# Autodesk Inventor assembly: Marina - simplificacion
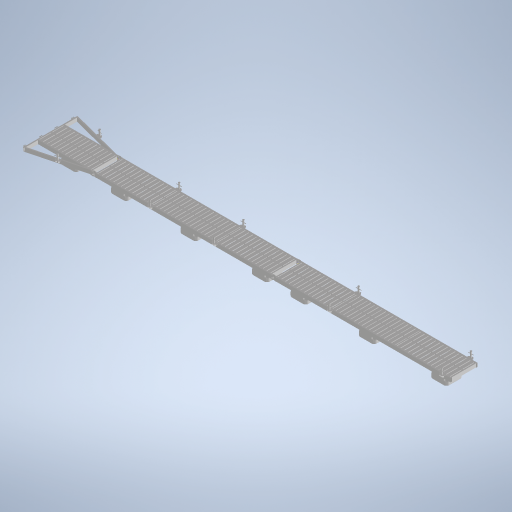
[picture p0: Inventor's stored thumbnail of the model, 512x512]
Saved by Autodesk Inventor 2023.2 (Build 272271000, 271)
## iProperties
Created: 2022-11-23
Part Number: Marina - simplificacion
Document SubType Name: Assembly
Designer: Maestria 1
Author: Maestria 1
## Documents named in this file (3)
- C:\Users\nekko\Documents\Modelos Orza SpA\Marina - simplificacion.iam
- C:\Users\nekko\Documents\Modelos Orza SpA\armazon.ipt
- C:\Users\nekko\Documents\Modelos Orza SpA\peldaño.ipt
## Components (103 placed, 2 different names)
1. armazon:1 — Nivelación:1, Coincidencia:1, Coincidencia:2, Nivelación:2, Coincidencia:3, Coincidencia:4, Coincidencia:5, Nivelación:3, Coincidencia:6, Mate:7, Flush:4, Mate:8, Flush:6, Flush:7, Mate:9, Flush:8, Mate:10, Flush:10, Flush:11, Mate:11, Flush:12, Mate:12, Flush:14, Flush:15, Mate:13, Flush:16, Mate:14, Flush:18, Flush:19, Flush:20, Mate:15, Mate:17, Flush:21, Flush:22, Mate:18, Flush:23
2. peldaño:2 — Nivelación:1, Coincidencia:1, Coincidencia:2
3. peldaño:1 — Nivelación:2, Coincidencia:3, Coincidencia:4
4. peldaño:15
5. peldaño:16
6. peldaño:17
7. peldaño:18
8. peldaño:19
9. peldaño:20
10. peldaño:21
11. peldaño:22
12. peldaño:23
13. peldaño:24
14. peldaño:25
15. peldaño:26
16. peldaño:3 — Mate:7, Flush:4, Flush:5
17. peldaño:4 — Coincidencia:5, Nivelación:3, Coincidencia:6, Flush:5
18. peldaño:27
19. peldaño:28
20. peldaño:29
21. peldaño:30
22. peldaño:31
23. peldaño:32
24. peldaño:33
25. peldaño:34
26. peldaño:35
27. peldaño:36
28. peldaño:37
29. peldaño:38
30. peldaño:7 — Mate:8, Flush:6, Flush:7, Flush:9
31. peldaño:6 — Mate:9, Flush:8, Flush:9
32. peldaño:39
33. peldaño:40
34. peldaño:41
35. peldaño:42
36. peldaño:43
37. peldaño:44
38. peldaño:45
39. peldaño:46
40. peldaño:47
41. peldaño:48
42. peldaño:49
43. peldaño:50
44. peldaño:51
45. peldaño:52
46. peldaño:5 — Mate:10, Flush:10, Flush:11, Flush:13
47. peldaño:8 — Mate:11, Flush:12, Flush:13
48. peldaño:53
49. peldaño:54
50. peldaño:55
51. peldaño:56
52. peldaño:57
53. peldaño:58
54. peldaño:59
55. peldaño:60
56. peldaño:61
57. peldaño:62
58. peldaño:63
59. peldaño:64
60. peldaño:9 — Mate:12, Flush:14, Flush:15, Flush:17
61. peldaño:10 — Mate:13, Flush:16, Flush:17
62. peldaño:65
63. peldaño:66
64. peldaño:67
65. peldaño:68
66. peldaño:69
67. peldaño:70
68. peldaño:71
69. peldaño:72
70. peldaño:73
71. peldaño:74
72. peldaño:75
73. peldaño:76
74. peldaño:11 — Flush:20, Mate:15, Mate:16
75. peldaño:12 — Mate:14, Flush:18, Flush:19, Mate:16
76. peldaño:77
77. peldaño:78
78. peldaño:79
79. peldaño:80
80. peldaño:81
81. peldaño:82
82. peldaño:83
83. peldaño:84
84. peldaño:85
85. peldaño:86
86. peldaño:87
87. peldaño:88
88. peldaño:89
89. peldaño:90
90. peldaño:13 — Mate:18, Flush:23, Flush:24
91. peldaño:14 — Mate:17, Flush:21, Flush:22, Flush:24
92. peldaño:91
93. peldaño:92
94. peldaño:93
95. peldaño:94
96. peldaño:95
97. peldaño:96
98. peldaño:97
99. peldaño:98
100. peldaño:99
101. peldaño:100
102. peldaño:101
103. peldaño:102
## Component patterns: (7 elements, first: peldaño:2 + peldaño:1), (7 elements, first: peldaño:3 + peldaño:4), (8 elements, first: peldaño:7 + peldaño:6), (7 elements, first: peldaño:5 + peldaño:8), (7 elements, first: peldaño:9 + peldaño:10), (8 elements, first: peldaño:11 + peldaño:12), (7 elements, first: peldaño:13 + peldaño:14)
## Relationships (42: Flush 24, Mate 18)
- Nivelación:1 [Flush]: armazon:1 ↔ peldaño:2
- Coincidencia:1 [Mate]: armazon:1 ↔ peldaño:2
- Coincidencia:2 [Mate] (25 mm): armazon:1 ↔ peldaño:2
- Nivelación:2 [Flush]: armazon:1 ↔ peldaño:1
- Coincidencia:3 [Mate]: armazon:1 ↔ peldaño:1
- Coincidencia:4 [Mate] (25 mm): armazon:1 ↔ peldaño:1
- Coincidencia:5 [Mate]: armazon:1 ↔ peldaño:4
- Nivelación:3 [Flush]: armazon:1 ↔ peldaño:4
- Coincidencia:6 [Mate] (25 mm): armazon:1 ↔ peldaño:4
- Mate:7: armazon:1 ↔ peldaño:3
- Flush:4: armazon:1 ↔ peldaño:3
- Flush:5: peldaño:3 ↔ peldaño:4
- Mate:8: armazon:1 ↔ peldaño:7
- Flush:6: armazon:1 ↔ peldaño:7
- Flush:7 (25 mm): armazon:1 ↔ peldaño:7
- Mate:9: armazon:1 ↔ peldaño:6
- Flush:8: armazon:1 ↔ peldaño:6
- Flush:9: peldaño:7 ↔ peldaño:6
- Mate:10: armazon:1 ↔ peldaño:5
- Flush:10: armazon:1 ↔ peldaño:5
- Flush:11 (25 mm): armazon:1 ↔ peldaño:5
- Mate:11: armazon:1 ↔ peldaño:8
- Flush:12: armazon:1 ↔ peldaño:8
- Flush:13: peldaño:5 ↔ peldaño:8
- Mate:12: armazon:1 ↔ peldaño:9
- Flush:14: armazon:1 ↔ peldaño:9
- Flush:15 (25 mm): armazon:1 ↔ peldaño:9
- Mate:13: armazon:1 ↔ peldaño:10
- Flush:16: armazon:1 ↔ peldaño:10
- Flush:17: peldaño:9 ↔ peldaño:10
- Mate:14: armazon:1 ↔ peldaño:12
- Flush:18: armazon:1 ↔ peldaño:12
- Flush:19 (25 mm): armazon:1 ↔ peldaño:12
- Flush:20: armazon:1 ↔ peldaño:11
- Mate:15: armazon:1 ↔ peldaño:11
- Mate:16: peldaño:11 ↔ peldaño:12
- Mate:17: armazon:1 ↔ peldaño:14
- Flush:21: armazon:1 ↔ peldaño:14
- Flush:22 (25 mm): armazon:1 ↔ peldaño:14
- Mate:18: armazon:1 ↔ peldaño:13
- Flush:23: armazon:1 ↔ peldaño:13
- Flush:24: peldaño:13 ↔ peldaño:14
